# Autodesk Inventor assembly: Coupler lift short + pulleys
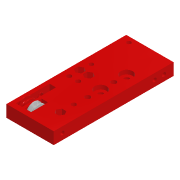
[picture p0: Inventor's stored thumbnail of the model, 180x180]
Saved by Autodesk Inventor 2020 (Build 240168000, 168)
## iProperties
Created: 2019-11-17
Part Number: Coupler lift short + pulleys
Document SubType Name: Assembly
Designer: ball
Author: ball
## Documents named in this file (4)
- C:\FTC\FTC8863CAD\2019 Robot\Delivery\Coupler lift short + pulleys.iam
- C:\FTC\FTC8863CAD\2019 Robot\Delivery\plastic pulley deep u.ipt
- C:\FTC\FTC8863CAD\RevRobotics\REV-41-1368 pulley.ipt
- C:\FTC\FTC8863CAD\2019 Robot\Delivery\Coupler lift short.ipt
## Components (3 placed, 3 different names)
1. Coupler lift short:1 — Mate:1, Mate:2, Mate:3, Mate:4
2. plastic pulley deep u:1 — Mate:1, Mate:2
3. REV-41-1368 pulley:1 — Mate:3, Mate:4
## Relationships (4: Mate 4)
- Mate:1: Coupler lift short:1 ↔ plastic pulley deep u:1
- Mate:2: Coupler lift short:1 ↔ plastic pulley deep u:1
- Mate:3: Coupler lift short:1 ↔ REV-41-1368 pulley:1
- Mate:4: Coupler lift short:1 ↔ REV-41-1368 pulley:1
